(part 1 of 2)
# Autodesk Inventor assembly: New Box ARm
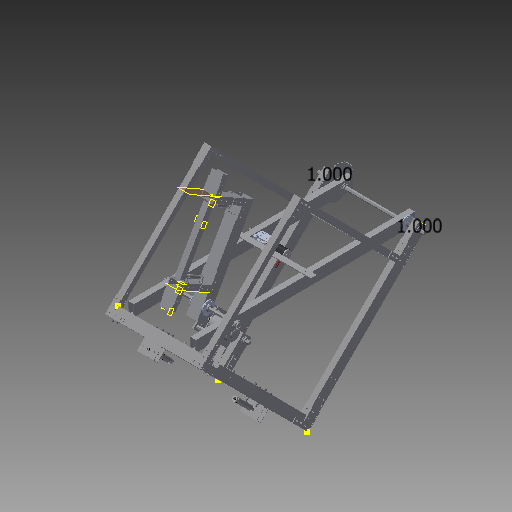
[picture p0: Inventor's stored thumbnail of the model, 512x512]
Saved by Autodesk Inventor 2018.3 (Build 223284000, 284)
## iProperties
Created: 2019-01-24
Part Number: New Box ARm
Document SubType Name: Assembly
Designer: Gabriel
Author: Gabriel
## Documents named in this file (36)
- C:\Users\Refraction\Documents\GitHub\2019CAD\Current Arm Box\New Box ARm.iam
- C:\Users\Refraction\Documents\GitHub\2019CAD\Current Arm Box\30in Vertical 1x2 Beam.ipt
- C:\Users\Refraction\Documents\GitHub\2019CAD\Current Arm Box\24in Vertical 1x1 Beam.ipt
- C:\Users\Refraction\Documents\GitHub\2019CAD\Current Arm Box\15in Horizontal 1x1 Beam.ipt
- C:\Users\Refraction\Documents\GitHub\2019CAD\Current Arm Box\24in Horizontal 1x1 Beam.ipt
- C:\Users\Refraction\Documents\GitHub\2019CAD\Current Arm Box\25in Horizontal 1x1 Beam.ipt
- C:\Users\Refraction\Documents\GitHub\2019CAD\Current Arm Box\ARm Gearbox.iam
- C:\Users\Refraction\Documents\GitHub\2019CAD\Current Arm Box\L gusset.ipt
- C:\Users\Refraction\Documents\GitHub\2019CAD\Current Arm Box\1_2_Acetal_Spacer_-_1_2_Hex_217-3261.ipt
- C:\Users\Refraction\Documents\GitHub\2019CAD\Current Arm Box\Clamping_Shaft_Collar_-_1_2_Hex_ID_217-2737.ipt
- C:\Users\Refraction\Documents\GitHub\2019CAD\Current Arm Box\_72t_Aluminum_Plate_Sprocket_25_Chain_1-1_8_Bearing_Bore_217-2627.ipt
- C:\Users\Refraction\Documents\GitHub\2019CAD\Current Arm Box\0_500_ID_x_1_125_OD_x_0_313_WD_Flanged_Bearing_217-2731.ipt
- C:\Users\Refraction\Documents\GitHub\2019CAD\Current Arm Box\41.75in Arm Beam Alternate (Right).ipt
- C:\Users\Refraction\Documents\GitHub\2019CAD\Current Arm Box\Hex Hub.ipt
- C:\Users\Refraction\Documents\GitHub\2019CAD\Current Arm Box\Hex Shaft ARm.ipt
- C:\Users\Refraction\Documents\GitHub\2019CAD\Current Arm Box\.75in 92196A245_18-8 STAINLESS STEEL SOCKET HEAD CAP SCREW.ipt
- C:\Users\Refraction\Documents\GitHub\2019CAD\Current Arm Box\1.5in 92196A251_18-8 STAINLESS STEEL SOCKET HEAD CAP SCREW.ipt
- C:\Users\Refraction\Documents\GitHub\2019CAD\Current Arm Box\LV Gusset.ipt
- C:\Users\Refraction\Documents\GitHub\2019CAD\Current Arm Box\am-3621 - S25-18HA-500H.ipt
- C:\Users\Refraction\Documents\GitHub\2019CAD\Current Arm Box\VersaPlanetary_v2_Two_Stage_100_1_with_BAG.ipt
- C:\Users\Refraction\Documents\GitHub\2019CAD\Current Arm Box\Wrist Hex Shaft 0.5in.ipt
- C:\Users\Refraction\Documents\GitHub\2019CAD\Current Arm Box\0_500_Hex_ID_x_1_125_OD_x_0_313_WD_Flanged_Bearing_v2_217-3875.ipt
- C:\Users\Refraction\Documents\GitHub\2019CAD\Current Arm Box\3D Model Spacer Arm.ipt
- C:\Users\Refraction\Documents\GitHub\2019CAD\Current Arm Box\92240A537_18-8 STAINLESS STEEL HEX HEAD CAP SCREW.ipt
- C:\Users\Refraction\Documents\GitHub\2019CAD\Current Arm Box\3D Model Washer Arm Gearbo.ipt
- C:\Users\Refraction\Documents\GitHub\2019CAD\Current Arm Box\1_16_Acetal_Spacer_-_1_2_Hex_217-3257.ipt
- C:\Users\Refraction\Documents\GitHub\2019CAD\Current Arm Box\41.75in Arm Beam Alternate (Left).ipt
- C:\Users\Refraction\Documents\GitHub\2019CAD\Drivebase but Calvin is a mad man\1x1 Bumper Attachment.ipt
- C:\Users\Refraction\Documents\GitHub\2019CAD\Drivebase but Calvin is a mad man\AIS2018\042.iam
- C:\Users\Refraction\Documents\GitHub\2019CAD\Drivebase but Calvin is a mad man\Arm Belly Pan.ipt
- C:\Users\Refraction\Documents\GitHub\2019CAD\Drivebase but Calvin is a mad man\73434-Fastenal-01-12-2019.ipt
- C:\Users\Refraction\Documents\GitHub\2019CAD\Drivebase but Calvin is a mad man\91831A011_TYPE 18-8 STAINLESS STL NYLON-INSERT LOCKNUT.ipt
- C:\Users\Refraction\Documents\GitHub\2019CAD\Current Arm Box\Gearbox Shaft Stabilizer.ipt
- C:\Users\Refraction\Documents\GitHub\2019CAD\Current Arm Box\1x2 L Bracket.ipt
- C:\Users\Refraction\Documents\GitHub\2019CAD\Current Arm Box\Hard Stop.ipt
- C:\Users\Refraction\Documents\GitHub\2019CAD\new Hatch design but everythig is broke\new Hatch design but everythig is broke\non integrated hatch.iam
## Components (169 placed, 35 different names)
1. 30in Vertical 1x2 Beam:1 — Mate:4, Mate:5, Mate:6, Flush:6, Flush:17, Mate:27, Mate:30, Flush:19, Flush:21, Flush:31, Mate:38, Mate:39, Flush:35, Mate:41, Flush:43, Flush:44, Mate:53, Mate:54, Mate:55, Mate:56, Mate:57, Flush:60, Mate:58, Mate:60, Mate:61, Mate:62, Flush:61, Mate:65, Mate:67, Mate:68, Mate:69, Flush:64, Mate:79, Mate:81, Mate:82, Mate:83, Flush:68, Mate:93, Mate:95, Mate:96, Mate:97, Flush:72, Mate:168, Mate:177, Mate:178, Mate:179, Flush:110, Flush:114, Flush:118, Mate:184, Mate:186, Mate:187, Mate:188, Flush:122, Flush:125, Mate:196, Mate:197, Mate:198, Mate:199
2. 30in Vertical 1x2 Beam:2 — Mate:7, Mate:8, Mate:9, Flush:5, Flush:18, Mate:33, Mate:35, Flush:25, Flush:27, Flush:31, Mate:37, Mate:40, Flush:34, Mate:47, Flush:49, Flush:50, Mate:72, Mate:74, Mate:75, Mate:76, Flush:66, Mate:86, Mate:88, Mate:89, Mate:90, Flush:70, Mate:100, Mate:102, Mate:103, Mate:104, Flush:74, Mate:107, Mate:109, Mate:110, Mate:111, Flush:76, Mate:170, Mate:172, Mate:173, Mate:174, Flush:112, Flush:116, Flush:117, Mate:182, Mate:191, Mate:192, Mate:193, Flush:120, Flush:126, Mate:200, Mate:201, Mate:202, Mate:203, Flush:144
3. 24in Vertical 1x1 Beam:3 — Flush:13, Flush:16, Flush:17, Mate:28, Mate:29, Flush:20, Flush:22, Flush:23, Mate:31, Flush:39, Mate:45, Mate:46, Flush:40, Mate:114, Flush:78, Flush:79, Mate:128, Flush:84, Flush:85, Mate:156, Mate:158, Mate:159, Flush:100, Flush:103, Mate:300, Mate:304, Mate:305, Flush:134, Flush:135
4. 24in Vertical 1x1 Beam:4 — Flush:16, Flush:18, Mate:32, Mate:34, Flush:24, Flush:26, Flush:32, Mate:36, Mate:51, Mate:52, Flush:46, Flush:47, Mate:121, Flush:81, Flush:82, Mate:135, Flush:87, Flush:88, Mate:162, Mate:164, Mate:165, Flush:105, Flush:108, Mate:306, Mate:310, Mate:311, Flush:130, Flush:131
5. 15in Horizontal 1x1 Beam:1 — Flush:13, Flush:30, Mate:42, Mate:43, Mate:44, Flush:41, Flush:42, Mate:48, Flush:45, Mate:49, Mate:50, Flush:48, Flush:52, Flush:53, Flush:56, Mate:157, Mate:160, Mate:161, Flush:99, Flush:101, Mate:163, Mate:166, Mate:167, Flush:104, Flush:106, Mate:242, Mate:509, Mate:510, Mate:511, Mate:516, Flush:141
6. 15in Horizontal 1x1 Beam:2 — Mate:4, Mate:5, Mate:6, Mate:7, Mate:8, Mate:9, Flush:5, Flush:6, Flush:30, Flush:38, Flush:54, Flush:55, Flush:56, Mate:169, Mate:171, Mate:175, Mate:176, Mate:180, Mate:181, Flush:109, Flush:111, Flush:113, Flush:115, Mate:506, Mate:507, Mate:508
7. 15in Horizontal 1x1 Beam:3 — Mate:37, Mate:38, Mate:39, Mate:40, Flush:34, Flush:35, Flush:36, Flush:37, Flush:38, Mate:183, Mate:185, Mate:189, Mate:190, Mate:194, Mate:195, Flush:119, Flush:121, Flush:123, Flush:124
8. 24in Horizontal 1x1 Beam:1 — Mate:32, Mate:33, Mate:34, Mate:35, Flush:24, Flush:25, Flush:26, Flush:27, Flush:32, Mate:36, Flush:33, Flush:37, Flush:58, Mate:73, Mate:77, Mate:78, Flush:65, Mate:87, Mate:91, Mate:92, Flush:69, Mate:122, Mate:123, Mate:124, Flush:80, Mate:136, Mate:137, Mate:138, Flush:86
9. 24in Horizontal 1x1 Beam:2 — Mate:27, Mate:28, Mate:29, Mate:30, Flush:19, Flush:20, Flush:21, Flush:22, Flush:23, Mate:31, Flush:33, Flush:36, Flush:57, Mate:66, Mate:70, Mate:71, Flush:63, Mate:80, Mate:84, Mate:85, Flush:67, Mate:115, Mate:116, Mate:117, Flush:77, Mate:129, Mate:130, Mate:131, Flush:83
10. 25in Horizontal 1x1 Beam:1 — Mate:41, Flush:39, Mate:42, Mate:43, Mate:44, Mate:45, Mate:46, Flush:40, Flush:41, Flush:42, Flush:43, Flush:44, Flush:51, Flush:53, Flush:55, Flush:57, Flush:59, Mate:59, Flush:62, Mate:94, Flush:71, Flush:102, Mate:301, Mate:302, Mate:303, Flush:133, Flush:136, Mate:560, Mate:561
11. 25in Horizontal 1x1 Beam:2 — Mate:47, Mate:48, Flush:45, Mate:49, Mate:50, Mate:51, Mate:52, Flush:46, Flush:47, Flush:48, Flush:49, Flush:50, Flush:51, Flush:52, Flush:54, Flush:58, Flush:59, Mate:101, Flush:73, Mate:108, Flush:75, Flush:107, Mate:307, Mate:308, Mate:309, Flush:129, Flush:132, Mate:554, Mate:555
12. ARm Gearbox:1 [sub-assembly] — Mate:53, Mate:54, Mate:55, Mate:56, Mate:57, Flush:60, Mate:575, Mate:576, Mate:581, Mate:582
13. L gusset:1 — Mate:93, Mate:94, Mate:95, Mate:96, Mate:97, Flush:71, Flush:72, Mate:517
14. L gusset:2 — Mate:100, Mate:101, Mate:102, Mate:103, Mate:104, Flush:73, Flush:74
15. L gusset:5 — Mate:114, Mate:115, Mate:116, Mate:117, Flush:77, Flush:78, Flush:79
16. L gusset:6 — Mate:121, Mate:122, Mate:123, Mate:124, Flush:80, Flush:81, Flush:82
17. L gusset:7 — Mate:72, Mate:73, Mate:74, Mate:75, Mate:76, Mate:77, Mate:78, Flush:65, Flush:66
18. L gusset:8 — Mate:65, Mate:66, Mate:67, Mate:68, Mate:69, Mate:70, Mate:71, Flush:63, Flush:64, Mate:273, Mate:274, Mate:275, Mate:277, Mate:289, Mate:291, Mate:292, Mate:293, Mate:382, Mate:383
19. L gusset:9 — Mate:58, Mate:59, Mate:60, Mate:61, Mate:62, Flush:61, Flush:62, Mate:259, Mate:260, Mate:261, Mate:263, Mate:285, Mate:286, Mate:287, Mate:288
20. L gusset:10 — Mate:107, Mate:108, Mate:109, Mate:110, Mate:111, Flush:75, Flush:76, Mate:296, Mate:297, Mate:298, Mate:328, Mate:329, Mate:330, Mate:337, Mate:338
21. L gusset:11 — Mate:86, Mate:87, Mate:88, Mate:89, Mate:90, Mate:91, Mate:92, Flush:69, Flush:70, Mate:364, Mate:365, Mate:366, Mate:368, Mate:369, Mate:370, Mate:372, Mate:373, Mate:380, Mate:381
22. L gusset:12 — Mate:79, Mate:80, Mate:81, Mate:82, Mate:83, Mate:84, Mate:85, Flush:67, Flush:68
23. L gusset:13 — Mate:135, Mate:136, Mate:137, Mate:138, Flush:86, Flush:87, Flush:88, Mate:332, Mate:333, Mate:334, Mate:335, Mate:336, Mate:359, Mate:360, Mate:361, Mate:362, Mate:363
24. L gusset:14 — Mate:128, Mate:129, Mate:130, Mate:131, Flush:83, Flush:84, Flush:85, Mate:268, Mate:269, Mate:270, Mate:271, Mate:272, Mate:278, Mate:279, Mate:280, Mate:281, Mate:282
25. L gusset:15 — Mate:168, Mate:169, Mate:177, Mate:178, Mate:179, Mate:180, Mate:181, Flush:109, Flush:110, Flush:113, Flush:114, Flush:118, Mate:339, Mate:340, Mate:341, Mate:342, Mate:349, Mate:350
26. L gusset:16 — Mate:156, Mate:157, Mate:158, Mate:159, Mate:160, Mate:161, Flush:99, Flush:100, Flush:101, Flush:102, Flush:103, Mate:351, Mate:352, Mate:357, Mate:358
27. L gusset:17 — Mate:184, Mate:185, Mate:186, Mate:187, Mate:188, Mate:189, Mate:190, Flush:121, Flush:122, Flush:123, Flush:125, Mate:376, Mate:377, Mate:388, Mate:389, Mate:390, Mate:391, Mate:394, Mate:395, Mate:400, Mate:401
28. L gusset:18 — Mate:162, Mate:163, Mate:164, Mate:165, Mate:166, Mate:167, Flush:104, Flush:105, Flush:106, Flush:107, Flush:108, Mate:353, Mate:354, Mate:355, Mate:356
29. L gusset:19 — Mate:170, Mate:171, Mate:172, Mate:173, Mate:174, Mate:175, Mate:176, Flush:111, Flush:112, Flush:115, Flush:116, Flush:117, Mate:343, Mate:344, Mate:345, Mate:346, Mate:347, Mate:348
30. L gusset:20 — Mate:182, Mate:183, Mate:191, Mate:192, Mate:193, Mate:194, Mate:195, Flush:119, Flush:120, Flush:124, Flush:126, Mate:384, Mate:385, Mate:386, Mate:387, Mate:392, Mate:393, Mate:396, Mate:397, Mate:398, Mate:399
31. 1_2_Acetal_Spacer_-_1_2_Hex_217-3261:1 — Mate:213, Mate:214, Mate:215, Mate:633
32. Clamping_Shaft_Collar_-_1_2_Hex_ID_217-2737:1 — Mate:204, Mate:205, Mate:641
33. _72t_Aluminum_Plate_Sprocket_25_Chain_1-1_8_Bearing_Bore_217-2627:1 — Mate:621, Mate:622, Mate:623, Mate:624, Mate:625
34. 0_500_ID_x_1_125_OD_x_0_313_WD_Flanged_Bearing_217-2731:1 — Mate:196, Mate:197
35. 41.75in Arm Beam Alternate (Right):1 — Mate:222, Mate:242, Mate:403, Mate:404, Mate:409, Mate:410, Mate:411, Mate:418, Mate:419, Mate:420, Mate:421, Mate:491, Mate:492, Mate:623, Mate:642
36. 0_500_ID_x_1_125_OD_x_0_313_WD_Flanged_Bearing_217-2731:2 — Mate:198, Mate:199, Mate:215
37. Hex Hub:2 — Mate:222, Mate:224, Mate:225, Rotation:4, Mate:621, Mate:622, Mate:624, Mate:625, Mate:634
38. Hex Shaft ARm:1 — Mate:204, Mate:205, Mate:213, Mate:214, Mate:224, Mate:225, Mate:230, Mate:231, Mate:236, Mate:237, Mate:240, Mate:241, Rotation:2, Rotation:4, Mate:631, Mate:632, Mate:635, Mate:636, Flush:144
39. Hex Hub:3 — Mate:240, Mate:241, Rotation:2, Mate:482, Mate:488, Mate:518, Mate:519, Mate:639
40. 1_2_Acetal_Spacer_-_1_2_Hex_217-3261:4 — Mate:230, Mate:231, Mate:232, Mate:638
41. 0_500_ID_x_1_125_OD_x_0_313_WD_Flanged_Bearing_217-2731:3 — Mate:201, Mate:203, Mate:232
42. 0_500_ID_x_1_125_OD_x_0_313_WD_Flanged_Bearing_217-2731:4 — Mate:200, Mate:202
43. Clamping_Shaft_Collar_-_1_2_Hex_ID_217-2737:2 — Mate:236, Mate:237, Mate:640
44. .75in 92196A245_18-8 STAINLESS STEEL SOCKET HEAD CAP SCREW:1 — Mate:376, Mate:377
45. 1.5in 92196A251_18-8 STAINLESS STEEL SOCKET HEAD CAP SCREW:1 — Mate:320, Mate:322
46. 1.5in 92196A251_18-8 STAINLESS STEEL SOCKET HEAD CAP SCREW:2 — Mate:317, Mate:319
47. 1.5in 92196A251_18-8 STAINLESS STEEL SOCKET HEAD CAP SCREW:3 — Mate:324, Mate:327
48. 1.5in 92196A251_18-8 STAINLESS STEEL SOCKET HEAD CAP SCREW:5 — Mate:341, Mate:350
49. 1.5in 92196A251_18-8 STAINLESS STEEL SOCKET HEAD CAP SCREW:6 — Mate:364, Mate:369
50. 1.5in 92196A251_18-8 STAINLESS STEEL SOCKET HEAD CAP SCREW:7 — Mate:312, Mate:315
51. 1.5in 92196A251_18-8 STAINLESS STEEL SOCKET HEAD CAP SCREW:8 — Mate:325, Mate:326
52. 1.5in 92196A251_18-8 STAINLESS STEEL SOCKET HEAD CAP SCREW:9 — Mate:271, Mate:281
53. 1.5in 92196A251_18-8 STAINLESS STEEL SOCKET HEAD CAP SCREW:10 — Mate:270, Mate:280
54. 1.5in 92196A251_18-8 STAINLESS STEEL SOCKET HEAD CAP SCREW:11 — Mate:313, Mate:314
55. 1.5in 92196A251_18-8 STAINLESS STEEL SOCKET HEAD CAP SCREW:12 — Mate:332, Mate:361
56. 1.5in 92196A251_18-8 STAINLESS STEEL SOCKET HEAD CAP SCREW:13 — Mate:259, Mate:288
57. .75in 92196A245_18-8 STAINLESS STEEL SOCKET HEAD CAP SCREW:14 — Mate:386, Mate:392
58. 1.5in 92196A251_18-8 STAINLESS STEEL SOCKET HEAD CAP SCREW:14 — Mate:316, Mate:318
59. .75in 92196A245_18-8 STAINLESS STEEL SOCKET HEAD CAP SCREW:15 — Mate:387, Mate:393
60. 1.5in 92196A251_18-8 STAINLESS STEEL SOCKET HEAD CAP SCREW:15 — Mate:297, Mate:329
61. .75in 92196A245_18-8 STAINLESS STEEL SOCKET HEAD CAP SCREW:17 — Mate:388, Mate:390
62. 1.5in 92196A251_18-8 STAINLESS STEEL SOCKET HEAD CAP SCREW:17 — Mate:298, Mate:330
63. 1.5in 92196A251_18-8 STAINLESS STEEL SOCKET HEAD CAP SCREW:18 — Mate:336, Mate:363
64. 1.5in 92196A251_18-8 STAINLESS STEEL SOCKET HEAD CAP SCREW:19 — Mate:366, Mate:372
65. 1.5in 92196A251_18-8 STAINLESS STEEL SOCKET HEAD CAP SCREW:20 — Mate:321, Mate:323
66. 1.5in 92196A251_18-8 STAINLESS STEEL SOCKET HEAD CAP SCREW:21 — Mate:339, Mate:340
67. 1.5in 92196A251_18-8 STAINLESS STEEL SOCKET HEAD CAP SCREW:22 — Mate:334, Mate:359
68. 1.5in 92196A251_18-8 STAINLESS STEEL SOCKET HEAD CAP SCREW:24 — Mate:261, Mate:286
69. 1.5in 92196A251_18-8 STAINLESS STEEL SOCKET HEAD CAP SCREW:25 — Mate:275, Mate:291
70. 1.5in 92196A251_18-8 STAINLESS STEEL SOCKET HEAD CAP SCREW:26 — Mate:333, Mate:360
71. 1.5in 92196A251_18-8 STAINLESS STEEL SOCKET HEAD CAP SCREW:27 — Mate:365, Mate:370
72. 1.5in 92196A251_18-8 STAINLESS STEEL SOCKET HEAD CAP SCREW:28 — Mate:337, Mate:338
73. 1.5in 92196A251_18-8 STAINLESS STEEL SOCKET HEAD CAP SCREW:30 — Mate:335, Mate:362
74. 1.5in 92196A251_18-8 STAINLESS STEEL SOCKET HEAD CAP SCREW:31 — Mate:368, Mate:373
75. 1.5in 92196A251_18-8 STAINLESS STEEL SOCKET HEAD CAP SCREW:33 — Mate:395, Mate:401
76. .75in 92196A245_18-8 STAINLESS STEEL SOCKET HEAD CAP SCREW:34 — Mate:384, Mate:385
77. 1.5in 92196A251_18-8 STAINLESS STEEL SOCKET HEAD CAP SCREW:34 — Mate:296, Mate:328
78. 1.5in 92196A251_18-8 STAINLESS STEEL SOCKET HEAD CAP SCREW:35 — Mate:273, Mate:293
79. 1.5in 92196A251_18-8 STAINLESS STEEL SOCKET HEAD CAP SCREW:36 — Mate:274, Mate:292
80. 1.5in 92196A251_18-8 STAINLESS STEEL SOCKET HEAD CAP SCREW:38 — Mate:263, Mate:287
81. 1.5in 92196A251_18-8 STAINLESS STEEL SOCKET HEAD CAP SCREW:39 — Mate:260, Mate:285
82. 1.5in 92196A251_18-8 STAINLESS STEEL SOCKET HEAD CAP SCREW:43 — Mate:277, Mate:289
83. 1.5in 92196A251_18-8 STAINLESS STEEL SOCKET HEAD CAP SCREW:45 — Mate:272, Mate:282
84. 1.5in 92196A251_18-8 STAINLESS STEEL SOCKET HEAD CAP SCREW:47 — Mate:269, Mate:278
85. 1.5in 92196A251_18-8 STAINLESS STEEL SOCKET HEAD CAP SCREW:49 — Mate:268, Mate:279
86. 1.5in 92196A251_18-8 STAINLESS STEEL SOCKET HEAD CAP SCREW:50 — Mate:397, Mate:399
87. 1.5in 92196A251_18-8 STAINLESS STEEL SOCKET HEAD CAP SCREW:51 — Mate:343, Mate:348
88. 1.5in 92196A251_18-8 STAINLESS STEEL SOCKET HEAD CAP SCREW:52 — Mate:342, Mate:349
89. 1.5in 92196A251_18-8 STAINLESS STEEL SOCKET HEAD CAP SCREW:54 — Mate:394, Mate:400
90. 1.5in 92196A251_18-8 STAINLESS STEEL SOCKET HEAD CAP SCREW:56 — Mate:396, Mate:398
91. LV Gusset:1 — Mate:306, Mate:307, Mate:308, Mate:309, Mate:310, Mate:311, Flush:129, Flush:130, Flush:131, Flush:132, Mate:320, Mate:321, Mate:322, Mate:323, Mate:324, Mate:325, Mate:326, Mate:327
92. LV Gusset:2 — Mate:300, Mate:301, Mate:302, Mate:303, Mate:304, Mate:305, Flush:133, Flush:134, Flush:135, Flush:136, Mate:312, Mate:313, Mate:314, Mate:315, Mate:316, Mate:317, Mate:318, Mate:319
93. 1.5in 92196A251_18-8 STAINLESS STEEL SOCKET HEAD CAP SCREW:58 — Mate:344, Mate:347
94. 1.5in 92196A251_18-8 STAINLESS STEEL SOCKET HEAD CAP SCREW:59 — Mate:345, Mate:346
95. 1.5in 92196A251_18-8 STAINLESS STEEL SOCKET HEAD CAP SCREW:60 — Mate:354, Mate:355
96. 1.5in 92196A251_18-8 STAINLESS STEEL SOCKET HEAD CAP SCREW:61 — Mate:352, Mate:358
97. 1.5in 92196A251_18-8 STAINLESS STEEL SOCKET HEAD CAP SCREW:64 — Mate:353, Mate:356
98. 1.5in 92196A251_18-8 STAINLESS STEEL SOCKET HEAD CAP SCREW:67 — Mate:351, Mate:357
99. 1.5in 92196A251_18-8 STAINLESS STEEL SOCKET HEAD CAP SCREW:68 — Mate:380, Mate:381
100. 1.5in 92196A251_18-8 STAINLESS STEEL SOCKET HEAD CAP SCREW:69 — Mate:382, Mate:383
101. .75in 92196A245_18-8 STAINLESS STEEL SOCKET HEAD CAP SCREW:58 — Mate:389, Mate:391
102. am-3621 - S25-18HA-500H:1 — Mate:422, Mate:423, Mate:424, Mate:428, Flush:140
103. 0_500_ID_x_1_125_OD_x_0_313_WD_Flanged_Bearing_217-2731:5 — Mate:449, Mate:494, Mate:495
104. 0_500_ID_x_1_125_OD_x_0_313_WD_Flanged_Bearing_217-2731:6 — Mate:403, Mate:409, Mate:447, Mate:459
105. 0_500_ID_x_1_125_OD_x_0_313_WD_Flanged_Bearing_217-2731:7 — Mate:404, Mate:410, Mate:453
106. 0_500_ID_x_1_125_OD_x_0_313_WD_Flanged_Bearing_217-2731:8 — Mate:460, Mate:493
107. VersaPlanetary_v2_Two_Stage_100_1_with_BAG:1 — Mate:419, Mate:420, Mate:421, Mate:422, Mate:423, Mate:426, Mate:427, Mate:429
108. am-3621 - S25-18HA-500H:2 — Mate:451, Mate:452, Mate:453, Flush:140
109. Wrist Hex Shaft 0.5in:1 — Mate:437, Mate:438, Flush:138, Mate:439, Mate:440, Mate:441, Mate:442, Mate:443, Mate:444, Mate:445, Mate:446, Mate:451, Mate:452, Mate:653, Mate:654, Mate:656, Mate:657, Mate:659, Mate:660
110. 0_500_Hex_ID_x_1_125_OD_x_0_313_WD_Flanged_Bearing_v2_217-3875:1 — Mate:411, Mate:418, Mate:424
111. 3D Model Spacer Arm:1 — Mate:426, Mate:427, Mate:428, Mate:431
112. 92240A537_18-8 STAINLESS STEEL HEX HEAD CAP SCREW:1 — Mate:429, Mate:430, Mate:432
113. 3D Model Washer Arm Gearbo:1 — Mate:430, Mate:431, Mate:432
114. Clamping_Shaft_Collar_-_1_2_Hex_ID_217-2737:4 — Mate:441, Mate:442, Mate:448, Mate:655
115. Clamping_Shaft_Collar_-_1_2_Hex_ID_217-2737:5 — Mate:439, Mate:440, Mate:450
116. Clamping_Shaft_Collar_-_1_2_Hex_ID_217-2737:6 — Mate:437, Mate:438, Flush:138, Mate:460, Mate:493
117. 1_16_Acetal_Spacer_-_1_2_Hex_217-3257:1 — Mate:445, Mate:446, Mate:447, Mate:448, Mate:459
118. 1_16_Acetal_Spacer_-_1_2_Hex_217-3257:2 — Mate:443, Mate:444, Mate:449, Mate:450
119. 0_500_ID_x_1_125_OD_x_0_313_WD_Flanged_Bearing_217-2731:9 — Mate:491, Mate:492, Mate:641
120. 0_500_ID_x_1_125_OD_x_0_313_WD_Flanged_Bearing_217-2731:10 — Mate:489, Mate:490, Mate:640
121. 41.75in Arm Beam Alternate (Left):1 — Mate:482, Mate:488, Mate:489, Mate:490, Mate:494, Mate:495, Mate:518, Mate:519, Mate:644
122. 1x1 Bumper Attachment:1 — Mate:509, Mate:510, Mate:511, Mate:514, Mate:515, Mate:530, Mate:532
123. 1x1 Bumper Attachment:2 — Mate:506, Mate:507, Mate:508, Mate:512, Mate:513, Mate:534, Mate:536
124. 042:1 [sub-assembly] — Mate:512, Mate:513
125. 042:2 [sub-assembly] — Mate:514, Mate:515
126. Arm Belly Pan:1 — Mate:516, Mate:517, Flush:141, Mate:522, Mate:523, Mate:524, Mate:525, Mate:526, Mate:527, Mate:528, Mate:529, Mate:538, Mate:539, Mate:540, Mate:541, Mate:542, Mate:543, Mate:544, Mate:545, Mate:546, Mate:547, Mate:548, Mate:549, Mate:550, Mate:551, Mate:552, Mate:553, Mate:556, Mate:557, Mate:558, Mate:559, Angle:1, Angle:2
127. 73434-Fastenal-01-12-2019:1 — Mate:523, Mate:525, Mate:535
128. 73434-Fastenal-01-12-2019:2 — Mate:522, Mate:524, Mate:537
129. 73434-Fastenal-01-12-2019:3 — Mate:527, Mate:528, Mate:531
130. 73434-Fastenal-01-12-2019:4 — Mate:526, Mate:529, Mate:533
131. 91831A011_TYPE 18-8 STAINLESS STL NYLON-INSERT LOCKNUT:1 — Mate:536, Mate:537
132. 91831A011_TYPE 18-8 STAINLESS STL NYLON-INSERT LOCKNUT:2 — Mate:534, Mate:535
133. 91831A011_TYPE 18-8 STAINLESS STL NYLON-INSERT LOCKNUT:3 — Mate:532, Mate:533
134. 91831A011_TYPE 18-8 STAINLESS STL NYLON-INSERT LOCKNUT:4 — Mate:530, Mate:531
135. 91831A011_TYPE 18-8 STAINLESS STL NYLON-INSERT LOCKNUT:5 — Mate:556, Mate:566
136. 91831A011_TYPE 18-8 STAINLESS STL NYLON-INSERT LOCKNUT:6 — Mate:554, Mate:569
137. 91831A011_TYPE 18-8 STAINLESS STL NYLON-INSERT LOCKNUT:7 — Mate:559, Mate:564
138. 91831A011_TYPE 18-8 STAINLESS STL NYLON-INSERT LOCKNUT:8 — Mate:558, Mate:565
139. 91831A011_TYPE 18-8 STAINLESS STL NYLON-INSERT LOCKNUT:9 — Mate:560, Mate:563
140. 91831A011_TYPE 18-8 STAINLESS STL NYLON-INSERT LOCKNUT:10 — Mate:561, Mate:562
141. 91831A011_TYPE 18-8 STAINLESS STL NYLON-INSERT LOCKNUT:11 — Mate:557, Mate:567
142. 91831A011_TYPE 18-8 STAINLESS STL NYLON-INSERT LOCKNUT:12 — Mate:555, Mate:568
143. 73434-Fastenal-01-12-2019:5 — Mate:543, Mate:553, Mate:568
144. 73434-Fastenal-01-12-2019:6 — Mate:542, Mate:552, Mate:569
145. 73434-Fastenal-01-12-2019:7 — Mate:545, Mate:546, Mate:562
146. 73434-Fastenal-01-12-2019:8 — Mate:544, Mate:547, Mate:563
147. 1.5in 92196A251_18-8 STAINLESS STEEL SOCKET HEAD CAP SCREW:70 — Mate:540, Mate:550, Mate:566
148. 1.5in 92196A251_18-8 STAINLESS STEEL SOCKET HEAD CAP SCREW:71 — Mate:541, Mate:551, Mate:567
149. 1.5in 92196A251_18-8 STAINLESS STEEL SOCKET HEAD CAP SCREW:72 — Mate:539, Mate:549, Mate:565
150. 1.5in 92196A251_18-8 STAINLESS STEEL SOCKET HEAD CAP SCREW:73 — Mate:538, Mate:548, Mate:564
151. Gearbox Shaft Stabilizer:1 — Mate:577, Mate:578, Mate:579, Mate:580, Angle:1, Mate:584, Mate:585, Mate:586, Mate:587, Mate:588, Mate:589, Mate:590, Mate:591
152. 0_500_ID_x_1_125_OD_x_0_313_WD_Flanged_Bearing_217-2731:11 — Mate:577, Mate:578, Mate:583, Mate:602, Mate:603
153. 0_500_ID_x_1_125_OD_x_0_313_WD_Flanged_Bearing_217-2731:12 — Mate:575, Mate:576, Mate:579, Mate:580, Mate:601, Mate:604
154. Clamping_Shaft_Collar_-_1_2_Hex_ID_217-2737:8 — Mate:581, Mate:582, Mate:583
155. 1x2 L Bracket:1 — Mate:584, Mate:585, Mate:586, Mate:587
156. 1x2 L Bracket:2 — Mate:588, Mate:589, Mate:590, Mate:591
157. Gearbox Shaft Stabilizer:2 — Mate:601, Mate:602, Mate:603, Mate:604, Angle:2, Mate:608, Mate:609, Mate:610, Mate:611, Mate:612, Mate:613
158. 1x2 L Bracket:3 — Mate:608, Mate:609, Mate:610, Mate:614, Mate:615, Mate:616, Mate:617
159. 1x2 L Bracket:4 — Mate:611, Mate:612, Mate:613
160. 1.5in 92196A251_18-8 STAINLESS STEEL SOCKET HEAD CAP SCREW:78 — Mate:615, Mate:616
161. 1.5in 92196A251_18-8 STAINLESS STEEL SOCKET HEAD CAP SCREW:79 — Mate:614, Mate:617
162. 1_2_Acetal_Spacer_-_1_2_Hex_217-3261:8 — Mate:631, Mate:632, Mate:633, Mate:634
163. 1_2_Acetal_Spacer_-_1_2_Hex_217-3261:10 — Mate:635, Mate:636, Mate:638, Mate:639
164. Hard Stop:1 — Mate:642, Mate:644
165. non integrated hatch:1 [sub-assembly] — Mate:645, Mate:646, Mate:647, Mate:648, Mate:649, Mate:650, Mate:651, Mate:652
166. Hex Hub:4 — Mate:645, Mate:650, Mate:651, Mate:652, Mate:653, Mate:654, Mate:655, Mate:658
167. Hex Hub:5 — Mate:646, Mate:647, Mate:648, Mate:649, Mate:661
168. Clamping_Shaft_Collar_-_1_2_Hex_ID_217-2737:9 — Mate:656, Mate:657, Mate:658
169. Clamping_Shaft_Collar_-_1_2_Hex_ID_217-2737:10 — Mate:659, Mate:660, Mate:661
## Relationships (581: Mate 463, Flush 114, RelateRotation 2, Angle 2)
- Mate:4: 30in Vertical 1x2 Beam:1 ↔ 15in Horizontal 1x1 Beam:2
- Mate:5: 30in Vertical 1x2 Beam:1 ↔ 15in Horizontal 1x1 Beam:2
- Mate:6: 30in Vertical 1x2 Beam:1 ↔ 15in Horizontal 1x1 Beam:2
- Mate:7: 30in Vertical 1x2 Beam:2 ↔ 15in Horizontal 1x1 Beam:2
- Mate:8: 30in Vertical 1x2 Beam:2 ↔ 15in Horizontal 1x1 Beam:2
- Mate:9: 30in Vertical 1x2 Beam:2 ↔ 15in Horizontal 1x1 Beam:2
- Flush:5: 30in Vertical 1x2 Beam:2 ↔ 15in Horizontal 1x1 Beam:2
- Flush:6: 30in Vertical 1x2 Beam:1 ↔ 15in Horizontal 1x1 Beam:2
- Flush:13: 24in Vertical 1x1 Beam:3 ↔ 15in Horizontal 1x1 Beam:1
- Flush:16: 24in Vertical 1x1 Beam:3 ↔ 24in Vertical 1x1 Beam:4
- Flush:17: 30in Vertical 1x2 Beam:1 ↔ 24in Vertical 1x1 Beam:3
- Flush:18: 30in Vertical 1x2 Beam:2 ↔ 24in Vertical 1x1 Beam:4
- Mate:27: 30in Vertical 1x2 Beam:1 ↔ 24in Horizontal 1x1 Beam:2
- Mate:28: 24in Vertical 1x1 Beam:3 ↔ 24in Horizontal 1x1 Beam:2
- Mate:29: 24in Vertical 1x1 Beam:3 ↔ 24in Horizontal 1x1 Beam:2
- Mate:30: 30in Vertical 1x2 Beam:1 ↔ 24in Horizontal 1x1 Beam:2
- Flush:19: 30in Vertical 1x2 Beam:1 ↔ 24in Horizontal 1x1 Beam:2
- Flush:20: 24in Vertical 1x1 Beam:3 ↔ 24in Horizontal 1x1 Beam:2
- Flush:21: 30in Vertical 1x2 Beam:1 ↔ 24in Horizontal 1x1 Beam:2
- Flush:22: 24in Vertical 1x1 Beam:3 ↔ 24in Horizontal 1x1 Beam:2
- Flush:23: 24in Vertical 1x1 Beam:3 ↔ 24in Horizontal 1x1 Beam:2
- Mate:31: 24in Vertical 1x1 Beam:3 ↔ 24in Horizontal 1x1 Beam:2
- Mate:32: 24in Vertical 1x1 Beam:4 ↔ 24in Horizontal 1x1 Beam:1
- Mate:33: 30in Vertical 1x2 Beam:2 ↔ 24in Horizontal 1x1 Beam:1
- Mate:34: 24in Vertical 1x1 Beam:4 ↔ 24in Horizontal 1x1 Beam:1
- Mate:35: 30in Vertical 1x2 Beam:2 ↔ 24in Horizontal 1x1 Beam:1
- Flush:24: 24in Vertical 1x1 Beam:4 ↔ 24in Horizontal 1x1 Beam:1
- Flush:25: 30in Vertical 1x2 Beam:2 ↔ 24in Horizontal 1x1 Beam:1
- Flush:26: 24in Vertical 1x1 Beam:4 ↔ 24in Horizontal 1x1 Beam:1
- Flush:27: 30in Vertical 1x2 Beam:2 ↔ 24in Horizontal 1x1 Beam:1
- Flush:30: 15in Horizontal 1x1 Beam:1 ↔ 15in Horizontal 1x1 Beam:2
- Flush:31: 30in Vertical 1x2 Beam:1 ↔ 30in Vertical 1x2 Beam:2
- Flush:32: 24in Vertical 1x1 Beam:4 ↔ 24in Horizontal 1x1 Beam:1
- Mate:36: 24in Vertical 1x1 Beam:4 ↔ 24in Horizontal 1x1 Beam:1
- Flush:33: 24in Horizontal 1x1 Beam:1 ↔ 24in Horizontal 1x1 Beam:2
- Mate:37: 30in Vertical 1x2 Beam:2 ↔ 15in Horizontal 1x1 Beam:3
- Mate:38: 30in Vertical 1x2 Beam:1 ↔ 15in Horizontal 1x1 Beam:3
- Mate:39: 30in Vertical 1x2 Beam:1 ↔ 15in Horizontal 1x1 Beam:3
- Mate:40: 30in Vertical 1x2 Beam:2 ↔ 15in Horizontal 1x1 Beam:3
- Flush:34: 30in Vertical 1x2 Beam:2 ↔ 15in Horizontal 1x1 Beam:3
- Flush:35: 30in Vertical 1x2 Beam:1 ↔ 15in Horizontal 1x1 Beam:3
- Flush:36: 15in Horizontal 1x1 Beam:3 ↔ 24in Horizontal 1x1 Beam:2
- Flush:37: 15in Horizontal 1x1 Beam:3 ↔ 24in Horizontal 1x1 Beam:1
- Flush:38: 15in Horizontal 1x1 Beam:2 ↔ 15in Horizontal 1x1 Beam:3
- Mate:41: 30in Vertical 1x2 Beam:1 ↔ 25in Horizontal 1x1 Beam:1
- Flush:39: 24in Vertical 1x1 Beam:3 ↔ 25in Horizontal 1x1 Beam:1
- Mate:42: 15in Horizontal 1x1 Beam:1 ↔ 25in Horizontal 1x1 Beam:1
- Mate:43: 15in Horizontal 1x1 Beam:1 ↔ 25in Horizontal 1x1 Beam:1
- Mate:44: 15in Horizontal 1x1 Beam:1 ↔ 25in Horizontal 1x1 Beam:1
- Mate:45: 24in Vertical 1x1 Beam:3 ↔ 25in Horizontal 1x1 Beam:1
- Mate:46: 24in Vertical 1x1 Beam:3 ↔ 25in Horizontal 1x1 Beam:1
- Flush:40: 24in Vertical 1x1 Beam:3 ↔ 25in Horizontal 1x1 Beam:1
- Flush:41: 15in Horizontal 1x1 Beam:1 ↔ 25in Horizontal 1x1 Beam:1
- Flush:42: 15in Horizontal 1x1 Beam:1 ↔ 25in Horizontal 1x1 Beam:1
- Flush:43: 30in Vertical 1x2 Beam:1 ↔ 25in Horizontal 1x1 Beam:1
- Flush:44: 30in Vertical 1x2 Beam:1 ↔ 25in Horizontal 1x1 Beam:1
- Mate:47: 30in Vertical 1x2 Beam:2 ↔ 25in Horizontal 1x1 Beam:2
- Mate:48: 15in Horizontal 1x1 Beam:1 ↔ 25in Horizontal 1x1 Beam:2
- Flush:45: 15in Horizontal 1x1 Beam:1 ↔ 25in Horizontal 1x1 Beam:2
- Mate:49: 15in Horizontal 1x1 Beam:1 ↔ 25in Horizontal 1x1 Beam:2
- Mate:50: 15in Horizontal 1x1 Beam:1 ↔ 25in Horizontal 1x1 Beam:2
- Mate:51: 24in Vertical 1x1 Beam:4 ↔ 25in Horizontal 1x1 Beam:2
- Mate:52: 24in Vertical 1x1 Beam:4 ↔ 25in Horizontal 1x1 Beam:2
- Flush:46: 24in Vertical 1x1 Beam:4 ↔ 25in Horizontal 1x1 Beam:2
- Flush:47: 24in Vertical 1x1 Beam:4 ↔ 25in Horizontal 1x1 Beam:2
- Flush:48: 15in Horizontal 1x1 Beam:1 ↔ 25in Horizontal 1x1 Beam:2
- Flush:49: 30in Vertical 1x2 Beam:2 ↔ 25in Horizontal 1x1 Beam:2
- Flush:50: 30in Vertical 1x2 Beam:2 ↔ 25in Horizontal 1x1 Beam:2
- Flush:51: 25in Horizontal 1x1 Beam:1 ↔ 25in Horizontal 1x1 Beam:2
- Flush:52: 15in Horizontal 1x1 Beam:1 ↔ 25in Horizontal 1x1 Beam:2
- Flush:53: 15in Horizontal 1x1 Beam:1 ↔ 25in Horizontal 1x1 Beam:1
- Flush:54: 15in Horizontal 1x1 Beam:2 ↔ 25in Horizontal 1x1 Beam:2
- Flush:55: 15in Horizontal 1x1 Beam:2 ↔ 25in Horizontal 1x1 Beam:1
- Flush:56: 15in Horizontal 1x1 Beam:1 ↔ 15in Horizontal 1x1 Beam:2
- Flush:57: 24in Horizontal 1x1 Beam:2 ↔ 25in Horizontal 1x1 Beam:1
- Flush:58: 24in Horizontal 1x1 Beam:1 ↔ 25in Horizontal 1x1 Beam:2
- Flush:59: 25in Horizontal 1x1 Beam:1 ↔ 25in Horizontal 1x1 Beam:2
- Mate:53: 30in Vertical 1x2 Beam:1 ↔ ARm Gearbox:1
- Mate:54: 30in Vertical 1x2 Beam:1 ↔ ARm Gearbox:1
- Mate:55: 30in Vertical 1x2 Beam:1 ↔ ARm Gearbox:1
- Mate:56: 30in Vertical 1x2 Beam:1 ↔ ARm Gearbox:1
- Mate:57: 30in Vertical 1x2 Beam:1 ↔ ARm Gearbox:1
- Flush:60: 30in Vertical 1x2 Beam:1 ↔ ARm Gearbox:1
- Mate:58: 30in Vertical 1x2 Beam:1 ↔ L gusset:9
- Mate:59: 25in Horizontal 1x1 Beam:1 ↔ L gusset:9
- Mate:60: 30in Vertical 1x2 Beam:1 ↔ L gusset:9
- Mate:61: 30in Vertical 1x2 Beam:1 ↔ L gusset:9
- Mate:62: 30in Vertical 1x2 Beam:1 ↔ L gusset:9
- Flush:61: 30in Vertical 1x2 Beam:1 ↔ L gusset:9
- Flush:62: 25in Horizontal 1x1 Beam:1 ↔ L gusset:9
- Mate:65: 30in Vertical 1x2 Beam:1 ↔ L gusset:8
- Mate:66: 24in Horizontal 1x1 Beam:2 ↔ L gusset:8
- Mate:67: 30in Vertical 1x2 Beam:1 ↔ L gusset:8
- Mate:68: 30in Vertical 1x2 Beam:1 ↔ L gusset:8
- Mate:69: 30in Vertical 1x2 Beam:1 ↔ L gusset:8
- Mate:70: 24in Horizontal 1x1 Beam:2 ↔ L gusset:8
- Mate:71: 24in Horizontal 1x1 Beam:2 ↔ L gusset:8
- Flush:63: 24in Horizontal 1x1 Beam:2 ↔ L gusset:8
- Flush:64: 30in Vertical 1x2 Beam:1 ↔ L gusset:8
- Mate:72: 30in Vertical 1x2 Beam:2 ↔ L gusset:7
- Mate:73: 24in Horizontal 1x1 Beam:1 ↔ L gusset:7
- Mate:74: 30in Vertical 1x2 Beam:2 ↔ L gusset:7
- Mate:75: 30in Vertical 1x2 Beam:2 ↔ L gusset:7
- Mate:76: 30in Vertical 1x2 Beam:2 ↔ L gusset:7
- Mate:77: 24in Horizontal 1x1 Beam:1 ↔ L gusset:7
- Mate:78: 24in Horizontal 1x1 Beam:1 ↔ L gusset:7
- Flush:65: 24in Horizontal 1x1 Beam:1 ↔ L gusset:7
- Flush:66: 30in Vertical 1x2 Beam:2 ↔ L gusset:7
- Mate:79: 30in Vertical 1x2 Beam:1 ↔ L gusset:12
- Mate:80: 24in Horizontal 1x1 Beam:2 ↔ L gusset:12
- Mate:81: 30in Vertical 1x2 Beam:1 ↔ L gusset:12
- Mate:82: 30in Vertical 1x2 Beam:1 ↔ L gusset:12
- Mate:83: 30in Vertical 1x2 Beam:1 ↔ L gusset:12
- Mate:84: 24in Horizontal 1x1 Beam:2 ↔ L gusset:12
- Mate:85: 24in Horizontal 1x1 Beam:2 ↔ L gusset:12
- Flush:67: 24in Horizontal 1x1 Beam:2 ↔ L gusset:12
- Flush:68: 30in Vertical 1x2 Beam:1 ↔ L gusset:12
- Mate:86: 30in Vertical 1x2 Beam:2 ↔ L gusset:11
- Mate:87: 24in Horizontal 1x1 Beam:1 ↔ L gusset:11
- Mate:88: 30in Vertical 1x2 Beam:2 ↔ L gusset:11
- Mate:89: 30in Vertical 1x2 Beam:2 ↔ L gusset:11
- Mate:90: 30in Vertical 1x2 Beam:2 ↔ L gusset:11
- Mate:91: 24in Horizontal 1x1 Beam:1 ↔ L gusset:11
- Mate:92: 24in Horizontal 1x1 Beam:1 ↔ L gusset:11
- Flush:69: 24in Horizontal 1x1 Beam:1 ↔ L gusset:11
- Flush:70: 30in Vertical 1x2 Beam:2 ↔ L gusset:11
- Mate:93: 30in Vertical 1x2 Beam:1 ↔ L gusset:1
- Mate:94: 25in Horizontal 1x1 Beam:1 ↔ L gusset:1
- Mate:95: 30in Vertical 1x2 Beam:1 ↔ L gusset:1
- Mate:96: 30in Vertical 1x2 Beam:1 ↔ L gusset:1
- Mate:97: 30in Vertical 1x2 Beam:1 ↔ L gusset:1
- Flush:71: 25in Horizontal 1x1 Beam:1 ↔ L gusset:1
- Flush:72: 30in Vertical 1x2 Beam:1 ↔ L gusset:1
- Mate:100: 30in Vertical 1x2 Beam:2 ↔ L gusset:2
- Mate:101: 25in Horizontal 1x1 Beam:2 ↔ L gusset:2
- Mate:102: 30in Vertical 1x2 Beam:2 ↔ L gusset:2
- Mate:103: 30in Vertical 1x2 Beam:2 ↔ L gusset:2
- Mate:104: 30in Vertical 1x2 Beam:2 ↔ L gusset:2
- Flush:73: 25in Horizontal 1x1 Beam:2 ↔ L gusset:2
- Flush:74: 30in Vertical 1x2 Beam:2 ↔ L gusset:2
- Mate:107: 30in Vertical 1x2 Beam:2 ↔ L gusset:10
- Mate:108: 25in Horizontal 1x1 Beam:2 ↔ L gusset:10
- Mate:109: 30in Vertical 1x2 Beam:2 ↔ L gusset:10
- Mate:110: 30in Vertical 1x2 Beam:2 ↔ L gusset:10
- Mate:111: 30in Vertical 1x2 Beam:2 ↔ L gusset:10
- Flush:75: 25in Horizontal 1x1 Beam:2 ↔ L gusset:10
- Flush:76: 30in Vertical 1x2 Beam:2 ↔ L gusset:10
- Mate:114: 24in Vertical 1x1 Beam:3 ↔ L gusset:5
- Mate:115: 24in Horizontal 1x1 Beam:2 ↔ L gusset:5
- Mate:116: 24in Horizontal 1x1 Beam:2 ↔ L gusset:5
- Mate:117: 24in Horizontal 1x1 Beam:2 ↔ L gusset:5
- Flush:77: 24in Horizontal 1x1 Beam:2 ↔ L gusset:5
- Flush:78: 24in Vertical 1x1 Beam:3 ↔ L gusset:5
- Flush:79: 24in Vertical 1x1 Beam:3 ↔ L gusset:5
- Mate:121: 24in Vertical 1x1 Beam:4 ↔ L gusset:6
- Mate:122: 24in Horizontal 1x1 Beam:1 ↔ L gusset:6
- Mate:123: 24in Horizontal 1x1 Beam:1 ↔ L gusset:6
- Mate:124: 24in Horizontal 1x1 Beam:1 ↔ L gusset:6
- Flush:80: 24in Horizontal 1x1 Beam:1 ↔ L gusset:6
- Flush:81: 24in Vertical 1x1 Beam:4 ↔ L gusset:6
- Flush:82: 24in Vertical 1x1 Beam:4 ↔ L gusset:6
- Mate:128: 24in Vertical 1x1 Beam:3 ↔ L gusset:14
- Mate:129: 24in Horizontal 1x1 Beam:2 ↔ L gusset:14
- Mate:130: 24in Horizontal 1x1 Beam:2 ↔ L gusset:14
- Mate:131: 24in Horizontal 1x1 Beam:2 ↔ L gusset:14
- Flush:83: 24in Horizontal 1x1 Beam:2 ↔ L gusset:14
- Flush:84: 24in Vertical 1x1 Beam:3 ↔ L gusset:14
- Flush:85: 24in Vertical 1x1 Beam:3 ↔ L gusset:14
- Mate:135: 24in Vertical 1x1 Beam:4 ↔ L gusset:13
- Mate:136: 24in Horizontal 1x1 Beam:1 ↔ L gusset:13
- Mate:137: 24in Horizontal 1x1 Beam:1 ↔ L gusset:13
- Mate:138: 24in Horizontal 1x1 Beam:1 ↔ L gusset:13
- Flush:86: 24in Horizontal 1x1 Beam:1 ↔ L gusset:13
- Flush:87: 24in Vertical 1x1 Beam:4 ↔ L gusset:13
- Flush:88: 24in Vertical 1x1 Beam:4 ↔ L gusset:13
- Mate:156: 24in Vertical 1x1 Beam:3 ↔ L gusset:16
- Mate:157: 15in Horizontal 1x1 Beam:1 ↔ L gusset:16
- Mate:158: 24in Vertical 1x1 Beam:3 ↔ L gusset:16
- Mate:159: 24in Vertical 1x1 Beam:3 ↔ L gusset:16
- Mate:160: 15in Horizontal 1x1 Beam:1 ↔ L gusset:16
- Mate:161: 15in Horizontal 1x1 Beam:1 ↔ L gusset:16
- Flush:99: 15in Horizontal 1x1 Beam:1 ↔ L gusset:16
- Flush:100: 24in Vertical 1x1 Beam:3 ↔ L gusset:16
- Flush:101: 15in Horizontal 1x1 Beam:1 ↔ L gusset:16
- Flush:102: 25in Horizontal 1x1 Beam:1 ↔ L gusset:16
- Flush:103: 24in Vertical 1x1 Beam:3 ↔ L gusset:16
- Mate:162: 24in Vertical 1x1 Beam:4 ↔ L gusset:18
- Mate:163: 15in Horizontal 1x1 Beam:1 ↔ L gusset:18
- Mate:164: 24in Vertical 1x1 Beam:4 ↔ L gusset:18
- Mate:165: 24in Vertical 1x1 Beam:4 ↔ L gusset:18
- Mate:166: 15in Horizontal 1x1 Beam:1 ↔ L gusset:18
- Mate:167: 15in Horizontal 1x1 Beam:1 ↔ L gusset:18
- Flush:104: 15in Horizontal 1x1 Beam:1 ↔ L gusset:18
- Flush:105: 24in Vertical 1x1 Beam:4 ↔ L gusset:18
- Flush:106: 15in Horizontal 1x1 Beam:1 ↔ L gusset:18
- Flush:107: 25in Horizontal 1x1 Beam:2 ↔ L gusset:18
- Flush:108: 24in Vertical 1x1 Beam:4 ↔ L gusset:18
- Mate:168: 30in Vertical 1x2 Beam:1 ↔ L gusset:15
- Mate:169: 15in Horizontal 1x1 Beam:2 ↔ L gusset:15
- Mate:170: 30in Vertical 1x2 Beam:2 ↔ L gusset:19
- Mate:171: 15in Horizontal 1x1 Beam:2 ↔ L gusset:19
- Mate:172: 30in Vertical 1x2 Beam:2 ↔ L gusset:19
- Mate:173: 30in Vertical 1x2 Beam:2 ↔ L gusset:19
- Mate:174: 30in Vertical 1x2 Beam:2 ↔ L gusset:19
- Mate:175: 15in Horizontal 1x1 Beam:2 ↔ L gusset:19
- Mate:176: 15in Horizontal 1x1 Beam:2 ↔ L gusset:19
- Mate:177: 30in Vertical 1x2 Beam:1 ↔ L gusset:15
- Mate:178: 30in Vertical 1x2 Beam:1 ↔ L gusset:15
- Mate:179: 30in Vertical 1x2 Beam:1 ↔ L gusset:15
- Mate:180: 15in Horizontal 1x1 Beam:2 ↔ L gusset:15
- Mate:181: 15in Horizontal 1x1 Beam:2 ↔ L gusset:15
- Flush:109: 15in Horizontal 1x1 Beam:2 ↔ L gusset:15
- Flush:110: 30in Vertical 1x2 Beam:1 ↔ L gusset:15
- Flush:111: 15in Horizontal 1x1 Beam:2 ↔ L gusset:19
- Flush:112: 30in Vertical 1x2 Beam:2 ↔ L gusset:19
- Flush:113: 15in Horizontal 1x1 Beam:2 ↔ L gusset:15
- Flush:114: 30in Vertical 1x2 Beam:1 ↔ L gusset:15
- Flush:115: 15in Horizontal 1x1 Beam:2 ↔ L gusset:19
- Flush:116: 30in Vertical 1x2 Beam:2 ↔ L gusset:19
- Flush:117: 30in Vertical 1x2 Beam:2 ↔ L gusset:19
- Flush:118: 30in Vertical 1x2 Beam:1 ↔ L gusset:15
- Mate:182: 30in Vertical 1x2 Beam:2 ↔ L gusset:20
- Mate:183: 15in Horizontal 1x1 Beam:3 ↔ L gusset:20
- Mate:184: 30in Vertical 1x2 Beam:1 ↔ L gusset:17
- Mate:185: 15in Horizontal 1x1 Beam:3 ↔ L gusset:17
- Mate:186: 30in Vertical 1x2 Beam:1 ↔ L gusset:17
- Mate:187: 30in Vertical 1x2 Beam:1 ↔ L gusset:17
- Mate:188: 30in Vertical 1x2 Beam:1 ↔ L gusset:17
- Mate:189: 15in Horizontal 1x1 Beam:3 ↔ L gusset:17
- Mate:190: 15in Horizontal 1x1 Beam:3 ↔ L gusset:17
- Mate:191: 30in Vertical 1x2 Beam:2 ↔ L gusset:20
- Mate:192: 30in Vertical 1x2 Beam:2 ↔ L gusset:20
- Mate:193: 30in Vertical 1x2 Beam:2 ↔ L gusset:20
- Mate:194: 15in Horizontal 1x1 Beam:3 ↔ L gusset:20
- Mate:195: 15in Horizontal 1x1 Beam:3 ↔ L gusset:20
- Flush:119: 15in Horizontal 1x1 Beam:3 ↔ L gusset:20
- Flush:120: 30in Vertical 1x2 Beam:2 ↔ L gusset:20
- Flush:121: 15in Horizontal 1x1 Beam:3 ↔ L gusset:17
- Flush:122: 30in Vertical 1x2 Beam:1 ↔ L gusset:17
- Flush:123: 15in Horizontal 1x1 Beam:3 ↔ L gusset:17
- Flush:124: 15in Horizontal 1x1 Beam:3 ↔ L gusset:20
- Flush:125: 30in Vertical 1x2 Beam:1 ↔ L gusset:17
- Flush:126: 30in Vertical 1x2 Beam:2 ↔ L gusset:20
- Mate:196: 30in Vertical 1x2 Beam:1 ↔ 0_500_ID_x_1_125_OD_x_0_313_WD_Flanged_Bearing_217-2731:1
- Mate:197: 30in Vertical 1x2 Beam:1 ↔ 0_500_ID_x_1_125_OD_x_0_313_WD_Flanged_Bearing_217-2731:1
- Mate:198: 30in Vertical 1x2 Beam:1 ↔ 0_500_ID_x_1_125_OD_x_0_313_WD_Flanged_Bearing_217-2731:2